# Autodesk Inventor assembly: base
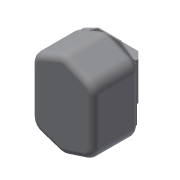
[picture p0: Inventor's stored thumbnail of the model, 180x180]
Saved by Autodesk Inventor 2014 SP1 (Build 180222100, 222)
## iProperties
Created: 2015-02-04
Part Number: base
Document SubType Name: Assembly
Designer: Simen
Author: Simen
## Documents named in this file (4)
- C:\Users\Simen\Documents\git\Eit\skjellet\base.iam
- C:\Users\Simen\Documents\git\Eit\skjellet\body.ipt
- C:\Users\Simen\Documents\git\Eit\skjellet\mount_bord.ipt
- C:\Users\Simen\Documents\git\Eit\skjellet\mount_holes_plate.ipt
## Components (3 placed, 3 different names)
1. body:1 — Mate:1, Mate:2, Flush:1, Mate:3, Flush:2
2. mount_bord:1 — Mate:1, Mate:2, Flush:1
3. mount_holes_plate:1 — Mate:3, Flush:2
## Relationships (5: Mate 3, Flush 2)
- Mate:1: body:1 ↔ mount_bord:1
- Mate:2: body:1 ↔ mount_bord:1
- Flush:1 (30 mm): body:1 ↔ mount_bord:1
- Mate:3: body:1 ↔ mount_holes_plate:1
- Flush:2 (30 mm): body:1 ↔ mount_holes_plate:1
